# Autodesk Inventor assembly: Pok Mk1
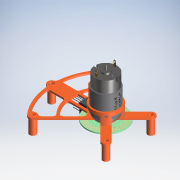
[picture p0: Inventor's stored thumbnail of the model, 180x180]
Saved by Autodesk Inventor 2018.2 (Build 222227000, 227)
## iProperties
Created: 2018-02-07
Part Number: Pok Mk1
Document SubType Name: Assembly
Designer: Moochster
Author: Moochster
## Documents named in this file (8)
- C:\Users\Moochster\OneDrive\Documents\2018 UBC\ELEC 391\Controller\CAD\Pok Mk1.iam
- C:\Users\Moochster\OneDrive\Documents\2018 UBC\ELEC 391\Controller\CAD\JD5B-2655W-R.ipt
- C:\Users\Moochster\OneDrive\Documents\2018 UBC\ELEC 391\Controller\CAD\Encoder Wheel (G16).ipt
- C:\Users\Moochster\OneDrive\Documents\2018 UBC\ELEC 391\Controller\CAD\Pok Yaw Motor Face Mount.ipt
- C:\Users\Moochster\OneDrive\Documents\2018 UBC\ELEC 391\Controller\CAD\Pok Washer I2mmO5mm.ipt
- C:\Users\Moochster\OneDrive\Documents\2018 UBC\ELEC 391\Controller\CAD\Shaft Washer.ipt
- C:\Users\Moochster\OneDrive\Documents\2018 UBC\ELEC 391\Controller\CAD\GP1A52HRJ00F (Large slot detector).ipt
- C:\Users\Moochster\OneDrive\Documents\2018 UBC\ELEC 391\Controller\CAD\Pok X-Carriage Bottom Support.ipt
## Components (13 placed, 7 different names)
1. JD5B-2655W-R:1 — Mate:1, Mate:2, Mate:4, Mate:7, Mate:8, Mate:11, Mate:24
2. Encoder Wheel (G16):1 — Mate:2, Mate:13, Mate:26, Mate:27, Angle:3
3. Pok Yaw Motor Face Mount:1 — Mate:4, Mate:5, Mate:6, Mate:9, Angle:1, Mate:20, Mate:21, Mate:22, Mate:23, Mate:24, Flush:3, Flush:4, Flush:5, Mate:25, Flush:7, Mate:26, Flush:8, Flush:9
4. Pok Washer I2mmO5mm:1 — Mate:6, Mate:7, Mate:9
5. Pok Washer I2mmO5mm:2 — Mate:5, Mate:8
6. Shaft Washer:1 — Mate:11, Mate:27, Angle:3
7. GP1A52HRJ00F (Large slot detector):1 — Mate:12, Flush:1, Flush:2, Mate:13
8. GP1A52HRJ00F (Large slot detector):2 — Mate:12, Flush:1, Flush:2, Angle:2
9. Pok X-Carriage Bottom Support:1 — Mate:23, Flush:8
10. Pok X-Carriage Bottom Support:2 — Mate:20, Mate:28, Flush:9
11. Pok X-Carriage Bottom Support:3 — Mate:22, Flush:5
12. Pok X-Carriage Bottom Support:4 — Mate:21, Flush:4
13. Pok X-Carriage Bottom Support:5 — Mate:25, Flush:7, Flush:3
## Relationships (31: Mate 20, Flush 8, Angle 3)
- Mate:1: JD5B-2655W-R:1
- Mate:2: JD5B-2655W-R:1 ↔ Encoder Wheel (G16):1
- Mate:4: JD5B-2655W-R:1 ↔ Pok Yaw Motor Face Mount:1
- Mate:5: Pok Yaw Motor Face Mount:1 ↔ Pok Washer I2mmO5mm:2
- Mate:6: Pok Yaw Motor Face Mount:1 ↔ Pok Washer I2mmO5mm:1
- Mate:7: JD5B-2655W-R:1 ↔ Pok Washer I2mmO5mm:1
- Mate:8: JD5B-2655W-R:1 ↔ Pok Washer I2mmO5mm:2
- Mate:9: Pok Yaw Motor Face Mount:1 ↔ Pok Washer I2mmO5mm:1
- Mate:11: JD5B-2655W-R:1 ↔ Shaft Washer:1
- Mate:12: GP1A52HRJ00F (Large slot detector):1 ↔ GP1A52HRJ00F (Large slot detector):2
- Flush:1: GP1A52HRJ00F (Large slot detector):1 ↔ GP1A52HRJ00F (Large slot detector):2
- Flush:2: GP1A52HRJ00F (Large slot detector):1 ↔ GP1A52HRJ00F (Large slot detector):2
- Mate:13 (0.7 mm): Encoder Wheel (G16):1 ↔ GP1A52HRJ00F (Large slot detector):1
- Angle:1 (0 deg): Pok Yaw Motor Face Mount:1
- Mate:20: Pok Yaw Motor Face Mount:1 ↔ Pok X-Carriage Bottom Support:2
- Mate:21: Pok Yaw Motor Face Mount:1 ↔ Pok X-Carriage Bottom Support:4
- Mate:22: Pok Yaw Motor Face Mount:1 ↔ Pok X-Carriage Bottom Support:3
- Mate:23: Pok Yaw Motor Face Mount:1 ↔ Pok X-Carriage Bottom Support:1
- Mate:24: JD5B-2655W-R:1 ↔ Pok Yaw Motor Face Mount:1
- Flush:3: Pok Yaw Motor Face Mount:1 ↔ Pok X-Carriage Bottom Support:5
- Flush:4: Pok Yaw Motor Face Mount:1 ↔ Pok X-Carriage Bottom Support:4
- Flush:5: Pok Yaw Motor Face Mount:1 ↔ Pok X-Carriage Bottom Support:3
- Mate:25: Pok Yaw Motor Face Mount:1 ↔ Pok X-Carriage Bottom Support:5
- Flush:7: Pok Yaw Motor Face Mount:1 ↔ Pok X-Carriage Bottom Support:5
- Angle:2 (0 deg): GP1A52HRJ00F (Large slot detector):2
- Mate:26 (1 mm): Encoder Wheel (G16):1 ↔ Pok Yaw Motor Face Mount:1
- Mate:27: Encoder Wheel (G16):1 ↔ Shaft Washer:1
- Mate:28: Pok X-Carriage Bottom Support:2
- Angle:3 (0 deg): Encoder Wheel (G16):1 ↔ Shaft Washer:1
- Flush:8: Pok Yaw Motor Face Mount:1 ↔ Pok X-Carriage Bottom Support:1
- Flush:9: Pok Yaw Motor Face Mount:1 ↔ Pok X-Carriage Bottom Support:2
